# Autodesk Inventor assembly: Clutch Bell
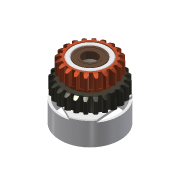
[picture p0: Inventor's stored thumbnail of the model, 180x180]
Saved by Autodesk Inventor 2022 Beta2 (Build 260130000, 130) ContinuousBuild 0
## iProperties
Shininess: 50.0
Length Units: 11269
Angle Units: 11279
Time Units: 11290
Mass Units: 11283
Length Display Precision: 4
Angle Display Precision: 2
Created: 2000-08-06
Part Number: Clutch Bell
Document SubType Name: Assembly
Designer: schneik
Density: 0.0
Volumn: 0.0
Area: 0.0
PropertySet Name: Model Information
Control State: 0
Master: False
Checked Out: False
Author: schneik
## Documents named in this file (5)
- C:\Autodesk Inventor 2021 Intro Practice Files\Clutch Bell.iam
- C:\Autodesk Inventor 2021 Intro Practice Files\Clutch Bearing.ipt
- C:\Autodesk Inventor 2021 Intro Practice Files\Clutch Bell.ipt
- C:\Autodesk Inventor 2021 Intro Practice Files\Clutch Gear 25t.ipt
- C:\Autodesk Inventor 2021 Intro Practice Files\Clutch Gear 20t.ipt
## Components (5 placed, 4 different names)
1. Clutch Bearing:1 — Insert:1
2. Clutch Bearing:2 — Insert:2
3. Clutch Bell:1 — Insert:1, Insert:2, Insert:3
4. Clutch Gear 24t.ipt:1 — Insert:3, Insert:4
5. Clutch Gear 20t:1 — Insert:4
## Relationships (4: Insert 4)
- Insert:1: Clutch Bearing:1 ↔ Clutch Bell:1
- Insert:2: Clutch Bearing:2 ↔ Clutch Bell:1
- Insert:3: Clutch Bell:1 ↔ Clutch Gear 24t.ipt:1
- Insert:4: Clutch Gear 24t.ipt:1 ↔ Clutch Gear 20t:1
